# Autodesk Inventor assembly: tractor
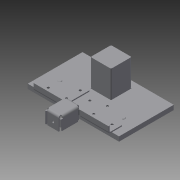
[picture p0: Inventor's stored thumbnail of the model, 180x180]
Saved by Autodesk Inventor 2013 (Build 170138000, 138)
## iProperties
Created: 2012-11-28
Part Number: tractor
Document SubType Name: Assembly
Designer: istvan.burbank
Author: istvan.burbank
## Documents named in this file (5)
- D:\GitHub\Crown-Fire\CAD\Frame\GantryMount\tractor.iam
- D:\GitHub\Crown-Fire\CAD\Frame\GantryMount\tractor.ipt
- D:\GitHub\Crown-Fire\CAD\Electronics\Motors\G723-280-4.ipt
- D:\GitHub\Crown-Fire\CAD\Hardware\Bearings\DualVee-size2.ipt
- D:\GitHub\Crown-Fire\CAD\Frame\GantryMount\gantryMount.ipt
## Components (5 placed, 4 different names)
1. tractor:1 — Mate:1, Mate:2, Mate:3, Mate:4, Mate:5, Mate:6, Mate:7, Mate:8
2. G723-280-4:1 — Mate:1, Mate:2, Mate:3
3. DualVee-size2:1 — Mate:5, Flush:1
4. DualVee-size2:2 — Mate:4, Flush:1
5. gantryMount:1 — Mate:6, Mate:7, Mate:8
## Relationships (9: Mate 8, Flush 1)
- Mate:1: tractor:1 ↔ G723-280-4:1
- Mate:2: tractor:1 ↔ G723-280-4:1
- Mate:3: tractor:1 ↔ G723-280-4:1
- Mate:4: tractor:1 ↔ DualVee-size2:2
- Mate:5: tractor:1 ↔ DualVee-size2:1
- Mate:6: tractor:1 ↔ gantryMount:1
- Mate:7: tractor:1 ↔ gantryMount:1
- Mate:8: tractor:1 ↔ gantryMount:1
- Flush:1: DualVee-size2:1 ↔ DualVee-size2:2
